# Autodesk Inventor assembly: ChestFrameDesign
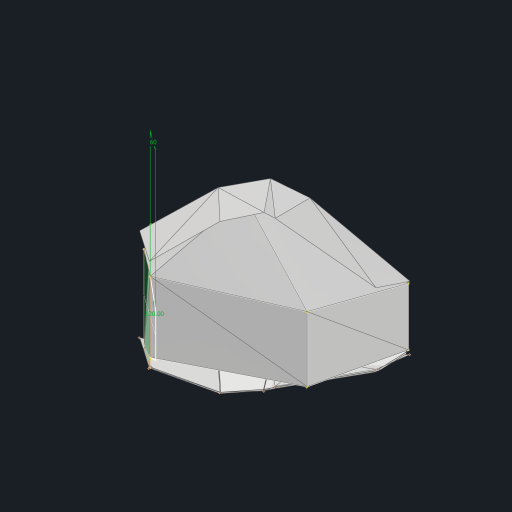
[picture p0: Inventor's stored thumbnail of the model, 512x512]
Saved by Autodesk Inventor 2023 (Build 270158000, 158)
## iProperties
Created: 2023-12-08
Part Number: ChestFrameDesign
Document SubType Name: Assembly
Designer: valer
_SolveAssemblyDoc: Frame Generator Solve Assembly
_Version: 15.0.0
Author: valer
## Documents named in this file (4)
- C:\Users\valer\Desktop\str1ker\design\ChestFrameDesign.iam
- C:\Users\valer\Desktop\str1ker\design\ChestFrameDesign.ipt
- C:\Users\valer\Desktop\str1ker\cad\Chest\Frame.iam
- C:\Users\valer\Desktop\str1ker\cad\chest\ChestSide.ipt
## Components (3 placed, 3 different names)
1. ChestFrameDesign:1 — Mate:1, Flush:1, Mate:2, Mate:3, Mate:4, Mate:5, Mate:6, Mate:7, Mate:8, Mate:9, Mate:10, Mate:11, Mate:12, Mate:13, Mate:14
2. Frame:1 [sub-assembly]
3. ChestSide:1 — Flush:1, Mate:12, Mate:13, Mate:14
## Relationships (15: Mate 14, Flush 1)
- Mate:1: ChestFrameDesign:1
- Flush:1: ChestFrameDesign:1 ↔ ChestSide:1
- Mate:2: ChestFrameDesign:1
- Mate:3: ChestFrameDesign:1
- Mate:4: ChestFrameDesign:1
- Mate:5: ChestFrameDesign:1
- Mate:6: ChestFrameDesign:1
- Mate:7: ChestFrameDesign:1
- Mate:8: ChestFrameDesign:1
- Mate:9: ChestFrameDesign:1
- Mate:10: ChestFrameDesign:1
- Mate:11: ChestFrameDesign:1
- Mate:12: ChestFrameDesign:1 ↔ ChestSide:1
- Mate:13: ChestFrameDesign:1 ↔ ChestSide:1
- Mate:14: ChestFrameDesign:1 ↔ ChestSide:1
